# Autodesk Inventor assembly: Left Angle Structure
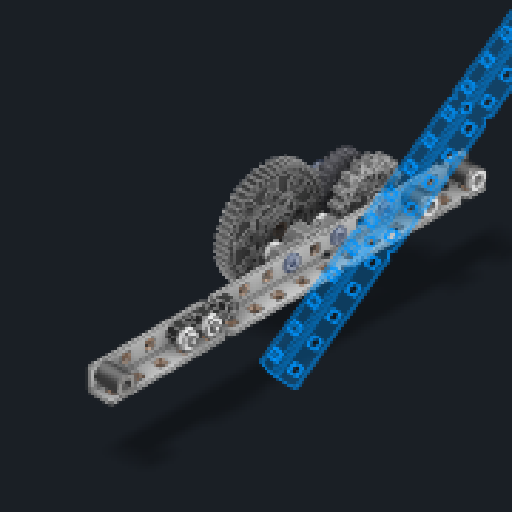
[picture p0: Inventor's stored thumbnail of the model, 512x512]
Saved by Autodesk Inventor 2025.1 (Build 291241000, 241)
## iProperties
Created: 2024-10-20
Part Number: Left Angle Structure
Document SubType Name: Assembly
Designer: Averey Ku
Author: Averey Ku
## Documents named in this file (18)
- C:\Users\avere\VEX\High Stakes\CAD\V2\Intake\Left Angle Structure.iam
- C:\Users\avere\VEX\High Stakes\CAD\ROBOPROS-CAD-Inventor\Motion\Spacers\Spacer Nylon .375 OD\NSpacer .375 OD x .375.ipt
- C:\Users\avere\VEX\High Stakes\CAD\ROBOPROS-CAD-Inventor\Motion\Spacers\Washer Steel\SWasher .375 OD x .062500.ipt
- C:\Users\avere\VEX\High Stakes\CAD\ROBOPROS-CAD-Inventor\Motion\Spacers\Washer Teflon\TWasher .375 OD x .04000.ipt
- C:\Users\avere\VEX\High Stakes\CAD\ROBOPROS-CAD-Inventor\Structure\Angle\Aluminum 1x1\Alu Angle 1x1x16.ipt
- C:\Users\avere\VEX\High Stakes\CAD\ROBOPROS-CAD-Inventor\Quick Assemblies\Bearing Flat NScrew Slotted Offset.iam
- C:\Users\avere\VEX\High Stakes\CAD\ROBOPROS-CAD-Inventor\Motion\Spacers\Spacer Nylon .375 OD\NSpacer .375 OD x .500.ipt
- C:\Users\avere\VEX\High Stakes\CAD\ROBOPROS-CAD-Inventor\Motion\Spacers\Washer Steel\SWasher .375 OD x .015625.ipt
- C:\Users\avere\VEX\High Stakes\CAD\ROBOPROS-CAD-Inventor\Motion\Shaft HS\HS Bearing Flat.ipt
- C:\Users\avere\VEX\High Stakes\CAD\ROBOPROS-CAD-Inventor\Structure\Hardware\Screw Shoulder Robosource\SScrew Shoulder Smooth .500 x .04.ipt
- C:\Users\avere\VEX\High Stakes\CAD\ROBOPROS-CAD-Inventor\Structure\Hardware\Nut Nylon\Nut Nylon - White.ipt
- C:\Users\avere\VEX\High Stakes\CAD\V2\Intake\Gearbox.iam
- Gearbox Left.iam
- C:\Users\avere\VEX\High Stakes\CAD\ROBOPROS-CAD-Inventor\Motion\Spacers\Spacer Nylon .375 OD.ipt
- C:\Users\avere\VEX\High Stakes\CAD\ROBOPROS-CAD-Inventor\Motion\Spacers\Washer Steel.ipt
- C:\Users\avere\VEX\High Stakes\CAD\ROBOPROS-CAD-Inventor\Structure\Hardware\Screw Shoulder Robosource.ipt
- C:\Users\avere\VEX\High Stakes\CAD\ROBOPROS-CAD-Inventor\Structure\Hardware\Nut Nylon.ipt
- C:\Users\avere\VEX\High Stakes\CAD\ROBOPROS-CAD-Inventor\Motion\Spacers\Washer Teflon.ipt
## Components (16 placed, 11 different names)
1. Alu Angle 1x1x16:1 — Flush:1, Mate:1, Mate:2, Insert:1, Mate:3, Insert:3, Insert:4, Mate:4, Insert:7, Insert:8, Insert:11, Insert:14, Insert:15
2. Bearing Flat NScrew Slotted Offset:1 [sub-assembly] — Insert:1, Mate:3
3. NSpacer .375 OD x .500:1 — Insert:2, Insert:3
4. SWasher .375 OD x .015625:1 — Insert:2
5. HS Bearing Flat:1 — Insert:4, Mate:4, Insert:5, Insert:6
6. SScrew Shoulder Smooth .500 x .04:1 — Insert:7
7. SScrew Shoulder Smooth .500 x .04:2 — Insert:8
8. Nut Nylon - White:1 — Insert:5
9. Nut Nylon - White:2 — Insert:6
10. NSpacer .375 OD x .375:2 — Insert:10, Insert:11
11. SWasher .375 OD x .062500:2 — Insert:9, Insert:10
12. TWasher .375 OD x .04000:1 — Insert:9
13. NSpacer .375 OD x .375:3 — Insert:14
14. SWasher .375 OD x .062500:3
15. TWasher .375 OD x .04000:2
16. Gearbox Left:1 [sub-assembly] — Insert:15
## Relationships (20: Insert 15, Mate 4, Flush 1)
- Flush:1 (-101.6 mm): Alu Angle 1x1x16:1
- Mate:1: Alu Angle 1x1x16:1
- Mate:2: Alu Angle 1x1x16:1
- Insert:1: Alu Angle 1x1x16:1 ↔ Bearing Flat NScrew Slotted Offset:1
- Mate:3: Alu Angle 1x1x16:1 ↔ Bearing Flat NScrew Slotted Offset:1
- Insert:2: NSpacer .375 OD x .500:1 ↔ SWasher .375 OD x .015625:1
- Insert:3: Alu Angle 1x1x16:1 ↔ NSpacer .375 OD x .500:1
- Insert:4: Alu Angle 1x1x16:1 ↔ HS Bearing Flat:1
- Mate:4: Alu Angle 1x1x16:1 ↔ HS Bearing Flat:1
- Insert:5: HS Bearing Flat:1 ↔ Nut Nylon - White:1
- Insert:6: HS Bearing Flat:1 ↔ Nut Nylon - White:2
- Insert:7: Alu Angle 1x1x16:1 ↔ SScrew Shoulder Smooth .500 x .04:1
- Insert:8: Alu Angle 1x1x16:1 ↔ SScrew Shoulder Smooth .500 x .04:2
- Insert:9: SWasher .375 OD x .062500:2 ↔ TWasher .375 OD x .04000:1
- Insert:10: NSpacer .375 OD x .375:2 ↔ SWasher .375 OD x .062500:2
- Insert:11: Alu Angle 1x1x16:1 ↔ NSpacer .375 OD x .375:2
- [Insert]: SWasher .375 OD x .062500:3 ↔ TWasher .375 OD x .04000:2
- [Insert]: NSpacer .375 OD x .375:3 ↔ SWasher .375 OD x .062500:3
- Insert:14: Alu Angle 1x1x16:1 ↔ NSpacer .375 OD x .375:3
- Insert:15 (3.175 mm): Alu Angle 1x1x16:1 ↔ Gearbox Left:1
## Named parameters: d40_d37 = 0 mm, d41_d38 = 0 mm
